# Autodesk Inventor assembly: 조립품1
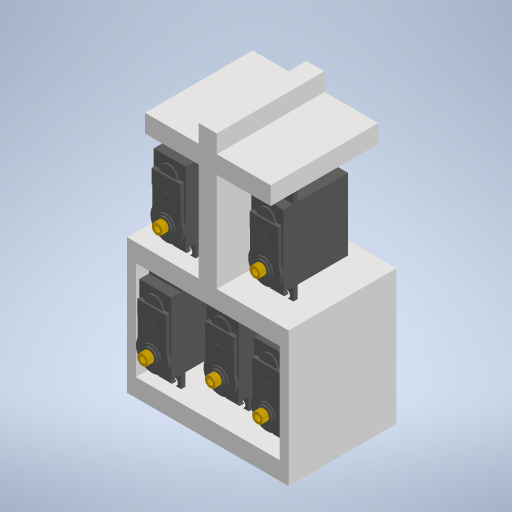
[picture p0: Inventor's stored thumbnail of the model, 512x512]
Saved by Autodesk Inventor 2024 (Build 280153000, 153)
## iProperties
Created: 2023-05-06
Part Number: 조립품1
Document SubType Name: Assembly
Designer: hjcho
Author: hjcho
## Documents named in this file (3)
- C:\Users\hjcho\Desktop\졸업작품\조립품1.iam
- C:\Users\hjcho\Desktop\졸업작품\팔.ipt
- C:\Users\hjcho\Desktop\졸업작품\Tower Pro MG996R.ipt
## Components (6 placed, 2 different names)
1. 팔:1 — 메이트:3, 메이트:5, 메이트:6, 메이트:7, 메이트:8, 메이트:9, 메이트:10, 메이트:11, 메이트:12, 메이트:13, 메이트:14, 메이트:15
2. Tower Pro MG996R:1 — 메이트:8, 메이트:9
3. Tower Pro MG996R:2 — 메이트:3, 메이트:5, 메이트:11, 메이트:12
4. Tower Pro MG996R:3 — 메이트:14, 메이트:15
5. Tower Pro MG996R:4 — 메이트:7, 메이트:13
6. Tower Pro MG996R:5 — 메이트:6, 메이트:10
## Relationships (12: Mate 12)
- 메이트:3 [Mate] (10 mm): 팔:1 ↔ Tower Pro MG996R:2
- 메이트:5 [Mate] (0.5 mm): 팔:1 ↔ Tower Pro MG996R:2
- 메이트:6 [Mate] (0.5 mm): 팔:1 ↔ Tower Pro MG996R:5
- 메이트:7 [Mate] (0.5 mm): 팔:1 ↔ Tower Pro MG996R:4
- 메이트:8 [Mate] (0.5 mm): 팔:1 ↔ Tower Pro MG996R:1
- 메이트:9 [Mate] (1 mm): 팔:1 ↔ Tower Pro MG996R:1
- 메이트:10 [Mate] (1 mm): 팔:1 ↔ Tower Pro MG996R:5
- 메이트:11 [Mate] (10 mm): 팔:1 ↔ Tower Pro MG996R:2
- 메이트:12 [Mate] (10 mm): 팔:1 ↔ Tower Pro MG996R:2
- 메이트:13 [Mate] (10 mm): 팔:1 ↔ Tower Pro MG996R:4
- 메이트:14 [Mate]: 팔:1 ↔ Tower Pro MG996R:3
- 메이트:15 [Mate] (1 mm): 팔:1 ↔ Tower Pro MG996R:3
